# Autodesk Inventor assembly: SEA Gearbox
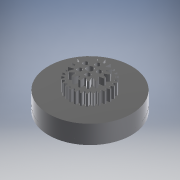
[picture p0: Inventor's stored thumbnail of the model, 180x180]
Saved by Autodesk Inventor 2017 (Build 210142000, 142)
## iProperties
Created: 2019-09-07
Part Number: SEA Gearbox
Document SubType Name: Assembly
Designer: Dell
Author: Dell
## Documents named in this file (5)
- C:\Users\Dell\Documents\GitHub\tr2\Actuator 1.6\SEA Gearbox.iam
- C:\Users\Dell\Documents\GitHub\tr2\Actuator 1.6\SE01.ipt
- C:\Users\Dell\Documents\GitHub\tr2\Actuator 1.6\SE02.ipt
- C:\Users\Dell\Documents\GitHub\tr2\Actuator 1.6\SE03.ipt
- C:\Users\Dell\Documents\GitHub\tr2\Actuator 1.6\SEA Gearbox\Design Accelerator\Spur Gears3.iam
## Components (4 placed, 4 different names)
1. SE01:1 — Mate:1, Mate:2, Mate:5, Mate:6
2. SE02:1 — Mate:1, Mate:2, Mate:3, Mate:4
3. SE03:1 — Mate:5, Mate:6
4. Spur Gears:1 [sub-assembly] — Mate:3, Mate:4
## Relationships (6: Mate 6)
- Mate:1: SE01:1 ↔ SE02:1
- Mate:2: SE01:1 ↔ SE02:1
- Mate:3: SE02:1 ↔ Spur Gears:1
- Mate:4: SE02:1 ↔ Spur Gears:1
- Mate:5: SE01:1 ↔ SE03:1
- Mate:6: SE01:1 ↔ SE03:1
